# Autodesk Inventor assembly: Stewart-Body-KST-DS215
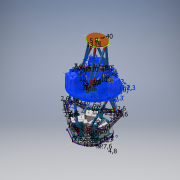
[picture p0: Inventor's stored thumbnail of the model, 180x180]
Saved by Autodesk Inventor 2018.2 (Build 222227000, 227)
## iProperties
Created: 2018-02-24
Part Number: Stewart-Body-KST-DS215
Material: Generisch
Document SubType Name: Assembly
Designer: JochenAlt
Author: JochenAlt
## Documents named in this file (8)
- D:\Projects\Donna\CAD\KST DS215MG\Donna-KST-DS215.iam
- D:\Projects\Donna\CAD\KST DS215MG\Stewart-Base-KST-DS215.iam
- D:\Projects\Donna\CAD\KST DS215MG\Servo-Arm-38mm-Ball-Joint.iam
- D:\Projects\Donna\CAD\KST DS215MG\Body-Rod-KST215MG.iam
- D:\Projects\Donna\CAD\KST DS215MG\Stewart-Body-KST215MG.iam
- D:\Projects\Donna\CAD\KST DS215MG\Servo-Arm-20mm-Ball-Joint.iam
- D:\Projects\Donna\CAD\KST DS215MG\Stewart-Head.iam
- D:\Projects\Donna\CAD\KST DS215MG\Head-Rod-KST215MG.iam
## Components (27 placed, 6 different names)
1. Stewart-Body:1 [sub-assembly] — Passend:1, Passend:2, Passend:3, Passend:4, Passend:5, Passend:6, Passend:7, Passend:8, Passend:9, Passend:10, Passend:11, Passend:12
2. Stewart-Body-Servo-Arm:1 [sub-assembly] — Passend:2, Passend:3, Passend:17
3. Stewart-Body-Servo-Arm:2 [sub-assembly] — Passend:1, Passend:4, Passend:16
4. Stewart-Body-Servo-Arm:3 [sub-assembly] — Passend:9, Passend:12, Passend:15
5. Stewart-Body-Servo-Arm:4 [sub-assembly] — Passend:10, Passend:11, Passend:13
6. Stewart-Body-Servo-Arm:5 [sub-assembly] — Passend:6, Passend:8, Passend:18
7. Stewart-Body-Servo-Arm:6 [sub-assembly] — Passend:5, Passend:7, Passend:14
8. BodyRod-KST215MG:1 [sub-assembly] — Passend:15, Passend:21
9. BodyRod-KST215MG:2 [sub-assembly] — Passend:13, Passend:22
10. BodyRod-KST215MG:3 [sub-assembly] — Passend:14, Passend:23
11. BodyRod-KST215MG:4 [sub-assembly] — Passend:18, Passend:24
12. BodyRod-KST215MG:5 [sub-assembly] — Passend:17, Passend:19
13. BodyRod-KST215MG:6 [sub-assembly] — Passend:16, Passend:20
14. Stewart-Body-KST215MG:1 [sub-assembly] — Passend:19, Passend:20, Passend:21, Passend:22, Passend:23, Passend:24, Passend:25, Passend:26, Passend:27, Passend:28, Passend:29, Passend:30, Passend:31, Passend:32, Passend:33, Passend:34, Passend:35, Passend:36
15. Servo-Arm-20mm-Ball-Joint:1 [sub-assembly] — Passend:25, Passend:30, Passend:39
16. Servo-Arm-20mm-Ball-Joint:2 [sub-assembly] — Passend:26, Passend:31, Passend:40
17. Servo-Arm-20mm-Ball-Joint:3 [sub-assembly] — Passend:27, Passend:32, Passend:42
18. Servo-Arm-20mm-Ball-Joint:4 [sub-assembly] — Passend:28, Passend:29, Passend:41
19. Servo-Arm-20mm-Ball-Joint:5 [sub-assembly] — Passend:33, Passend:36, Passend:37
20. Servo-Arm-20mm-Ball-Joint:6 [sub-assembly] — Passend:34, Passend:35, Passend:38
21. Stewart-Head:1 [sub-assembly] — Passend:43, Passend:44, Passend:45, Passend:46, Passend:47, Passend:48
22. BodyRod-KST215MG:7 [sub-assembly] — Passend:39, Passend:43
23. BodyRod-KST215MG:8 [sub-assembly] — Passend:40, Passend:44
24. BodyRod-KST215MG:9 [sub-assembly] — Passend:41, Passend:47
25. BodyRod-KST215MG:10 [sub-assembly] — Passend:42, Passend:48
26. BodyRod-KST215MG:11 [sub-assembly] — Passend:38, Passend:46
27. BodyRod-KST215MG:12 [sub-assembly] — Passend:37, Passend:45
## Relationships (48: Mate 48)
- Passend:1 [Mate]: Stewart-Body:1 ↔ Stewart-Body-Servo-Arm:2
- Passend:2 [Mate]: Stewart-Body:1 ↔ Stewart-Body-Servo-Arm:1
- Passend:3 [Mate]: Stewart-Body:1 ↔ Stewart-Body-Servo-Arm:1
- Passend:4 [Mate]: Stewart-Body:1 ↔ Stewart-Body-Servo-Arm:2
- Passend:5 [Mate]: Stewart-Body:1 ↔ Stewart-Body-Servo-Arm:6
- Passend:6 [Mate]: Stewart-Body:1 ↔ Stewart-Body-Servo-Arm:5
- Passend:7 [Mate]: Stewart-Body:1 ↔ Stewart-Body-Servo-Arm:6
- Passend:8 [Mate]: Stewart-Body:1 ↔ Stewart-Body-Servo-Arm:5
- Passend:9 [Mate]: Stewart-Body:1 ↔ Stewart-Body-Servo-Arm:3
- Passend:10 [Mate]: Stewart-Body:1 ↔ Stewart-Body-Servo-Arm:4
- Passend:11 [Mate]: Stewart-Body:1 ↔ Stewart-Body-Servo-Arm:4
- Passend:12 [Mate]: Stewart-Body:1 ↔ Stewart-Body-Servo-Arm:3
- Passend:13 [Mate]: Stewart-Body-Servo-Arm:4 ↔ BodyRod-KST215MG:2
- Passend:14 [Mate]: Stewart-Body-Servo-Arm:6 ↔ BodyRod-KST215MG:3
- Passend:15 [Mate]: Stewart-Body-Servo-Arm:3 ↔ BodyRod-KST215MG:1
- Passend:16 [Mate]: Stewart-Body-Servo-Arm:2 ↔ BodyRod-KST215MG:6
- Passend:17 [Mate]: Stewart-Body-Servo-Arm:1 ↔ BodyRod-KST215MG:5
- Passend:18 [Mate]: Stewart-Body-Servo-Arm:5 ↔ BodyRod-KST215MG:4
- Passend:19 [Mate]: BodyRod-KST215MG:5 ↔ Stewart-Body-KST215MG:1
- Passend:20 [Mate]: BodyRod-KST215MG:6 ↔ Stewart-Body-KST215MG:1
- Passend:21 [Mate]: BodyRod-KST215MG:1 ↔ Stewart-Body-KST215MG:1
- Passend:22 [Mate]: BodyRod-KST215MG:2 ↔ Stewart-Body-KST215MG:1
- Passend:23 [Mate]: BodyRod-KST215MG:3 ↔ Stewart-Body-KST215MG:1
- Passend:24 [Mate]: BodyRod-KST215MG:4 ↔ Stewart-Body-KST215MG:1
- Passend:25 [Mate]: Stewart-Body-KST215MG:1 ↔ Servo-Arm-20mm-Ball-Joint:1
- Passend:26 [Mate]: Stewart-Body-KST215MG:1 ↔ Servo-Arm-20mm-Ball-Joint:2
- Passend:27 [Mate]: Stewart-Body-KST215MG:1 ↔ Servo-Arm-20mm-Ball-Joint:3
- Passend:28 [Mate]: Stewart-Body-KST215MG:1 ↔ Servo-Arm-20mm-Ball-Joint:4
- Passend:29 [Mate]: Stewart-Body-KST215MG:1 ↔ Servo-Arm-20mm-Ball-Joint:4
- Passend:30 [Mate]: Stewart-Body-KST215MG:1 ↔ Servo-Arm-20mm-Ball-Joint:1
- Passend:31 [Mate]: Stewart-Body-KST215MG:1 ↔ Servo-Arm-20mm-Ball-Joint:2
- Passend:32 [Mate]: Stewart-Body-KST215MG:1 ↔ Servo-Arm-20mm-Ball-Joint:3
- Passend:33 [Mate]: Stewart-Body-KST215MG:1 ↔ Servo-Arm-20mm-Ball-Joint:5
- Passend:34 [Mate]: Stewart-Body-KST215MG:1 ↔ Servo-Arm-20mm-Ball-Joint:6
- Passend:35 [Mate]: Stewart-Body-KST215MG:1 ↔ Servo-Arm-20mm-Ball-Joint:6
- Passend:36 [Mate]: Stewart-Body-KST215MG:1 ↔ Servo-Arm-20mm-Ball-Joint:5
- Passend:37 [Mate]: Servo-Arm-20mm-Ball-Joint:5 ↔ BodyRod-KST215MG:12
- Passend:38 [Mate]: Servo-Arm-20mm-Ball-Joint:6 ↔ BodyRod-KST215MG:11
- Passend:39 [Mate]: Servo-Arm-20mm-Ball-Joint:1 ↔ BodyRod-KST215MG:7
- Passend:40 [Mate]: Servo-Arm-20mm-Ball-Joint:2 ↔ BodyRod-KST215MG:8
- Passend:41 [Mate]: Servo-Arm-20mm-Ball-Joint:4 ↔ BodyRod-KST215MG:9
- Passend:42 [Mate]: Servo-Arm-20mm-Ball-Joint:3 ↔ BodyRod-KST215MG:10
- Passend:43 [Mate]: Stewart-Head:1 ↔ BodyRod-KST215MG:7
- Passend:44 [Mate]: Stewart-Head:1 ↔ BodyRod-KST215MG:8
- Passend:45 [Mate]: Stewart-Head:1 ↔ BodyRod-KST215MG:12
- Passend:46 [Mate]: Stewart-Head:1 ↔ BodyRod-KST215MG:11
- Passend:47 [Mate]: Stewart-Head:1 ↔ BodyRod-KST215MG:9
- Passend:48 [Mate]: Stewart-Head:1 ↔ BodyRod-KST215MG:10
